# Autodesk Inventor assembly: Puzzle Cube Assembly
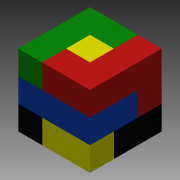
[picture p0: Inventor's stored thumbnail of the model, 180x180]
Saved by Autodesk Inventor 2015 (Build 190159000, 159)
## iProperties
Created: 2017-11-16
Part Number: Puzzle Cube Assembly
Document SubType Name: Assembly
Designer: Administrator
Author: Administrator
## Documents named in this file (6)
- L:\IED 9th\Puzzle Cube\Puzzle Cube Assembly.iam
- L:\IED 9th\Puzzle Cube\Yellow Puzzle Cube.ipt
- L:\IED 9th\Puzzle Cube\Black Puzzle Cube.ipt
- L:\IED 9th\Puzzle Cube\Blue Puzzle Cube.ipt
- L:\IED 9th\Puzzle Cube\Red Puzzle Cube.ipt
- L:\IED 9th\Puzzle Cube\Green Puzzle Cube.ipt
## Components (5 placed, 5 different names)
1. Yellow Puzzle Cube:1 — Mate:1, Flush:1, Flush:2, Mate:2, Flush:4, Flush:5
2. Black Puzzle Cube:1 — Mate:1, Flush:1, Flush:2, Mate:2, Mate:3, Flush:3, Mate:4, Flush:6, Flush:7
3. Blue Puzzle Cube:1 — Mate:3, Flush:3, Flush:4
4. Red Puzzle Cube:1 — Mate:4, Flush:5, Flush:6, Flush:7, Mate:5, Flush:8, Flush:9
5. Green Puzzle Cube:1 — Mate:5, Flush:8, Flush:9
## Relationships (14: Flush 9, Mate 5)
- Mate:1: Yellow Puzzle Cube:1 ↔ Black Puzzle Cube:1
- Flush:1: Yellow Puzzle Cube:1 ↔ Black Puzzle Cube:1
- Flush:2: Yellow Puzzle Cube:1 ↔ Black Puzzle Cube:1
- Mate:2: Yellow Puzzle Cube:1 ↔ Black Puzzle Cube:1
- Mate:3: Black Puzzle Cube:1 ↔ Blue Puzzle Cube:1
- Flush:3: Black Puzzle Cube:1 ↔ Blue Puzzle Cube:1
- Flush:4: Yellow Puzzle Cube:1 ↔ Blue Puzzle Cube:1
- Mate:4: Black Puzzle Cube:1 ↔ Red Puzzle Cube:1
- Flush:5: Yellow Puzzle Cube:1 ↔ Red Puzzle Cube:1
- Flush:6: Black Puzzle Cube:1 ↔ Red Puzzle Cube:1
- Flush:7: Black Puzzle Cube:1 ↔ Red Puzzle Cube:1
- Mate:5: Red Puzzle Cube:1 ↔ Green Puzzle Cube:1
- Flush:8: Red Puzzle Cube:1 ↔ Green Puzzle Cube:1
- Flush:9: Red Puzzle Cube:1 ↔ Green Puzzle Cube:1
